# Autodesk Inventor assembly: Сборка част.-аналог.V3.0
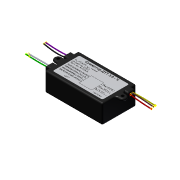
[picture p0: Inventor's stored thumbnail of the model, 180x180]
Saved by Autodesk Inventor 2012 (Build 160160000, 160)
## iProperties
Created: 2009-11-20
Part Number: Сборка част.-аналог.V3.0
Document SubType Name: Assembly
Designer: toma
Mass: 20.6369 g
Surface Area: 289.802 cm^2
Volume: 20.6369 cm^3
Density: 1 g/cm^3
Author: toma
## Documents named in this file (7)
- D:\VSS_WORK\VSS_ENERGO\Сумматор light\КД\Сумматор Light\Сумматор частотно-аналоговый\Сборка част.-аналог.V3.0.iam
- D:\VSS_WORK\VSS_ENERGO\Сумматор light\КД\Сумматор Light\корпус.ipt
- D:\VSS_WORK\VSS_ENERGO\Сумматор light\КД\Сумматор Light\клей.ipt
- D:\VSS_WORK\VSS_ENERGO\Сумматор light\КД\Сумматор Light\контакт.ipt
- D:\Inventor\Сумматор Light\Сборка2\AIP\Провода и кабели\Сборка2.Прокладка кабелей1.iam
- D:\VSS_WORK\VSS_ENERGO\Сумматор light\КД\Сумматор Light\Импортированные компоненты\Сумматор light частотно-аналоговый V3.0\Сумматор light частотно-аналоговый V3.0.iam
- D:\VSS_WORK\VSS_ENERGO\Сумматор light\КД\Сумматор Light\Сумматор частотно-аналоговый\крышка Ч_А.ipt
## Components (20 placed, 6 different names)
1. корпус:1 — Совмещение:4, Совмещение:5, Совмещение:6, Совмещение:8, Совмещение:9, Совмещение:10, Совмещение:11, Совмещение:12, Совмещение:13, Совмещение:14, Совмещение:17, Совмещение:18, Совмещение:19, Совмещение:20, Совмещение:21, Совмещение:22, Совмещение:23, Совмещение:24, Совмещение:25, Совмещение:26, Совмещение:27, Совмещение:28, Совмещение:38, Совмещение:41, Совмещение:42, Совмещение:43, Совмещение:44, Совмещение:45, Совмещение:47, Совмещение:48, Совмещение:49
2. клей:1 — Совмещение:4, Совмещение:39, Совмещение:40, Совмещение:41, Совмещение:42
3. контакт:1 — Совмещение:5, Совмещение:6, Совмещение:11
4. контакт:2 — Совмещение:8, Совмещение:9, Совмещение:10
5. контакт:3 — Совмещение:12, Совмещение:13, Совмещение:14
6. контакт:4 — Совмещение:18, Совмещение:19, Совмещение:20
7. контакт:5 — Совмещение:17, Совмещение:21, Совмещение:22
8. контакт:6 — Совмещение:23, Совмещение:24, Совмещение:25
9. контакт:7 — Совмещение:26, Совмещение:27, Совмещение:28
10. Прокладка кабелей1 [sub-assembly]
11. Сумматор light частотно-аналоговый V3.0:1 [sub-assembly] — Совмещение:38, Совмещение:39, Совмещение:40
12. контакт:8
13. контакт:9
14. контакт:10
15. контакт:11
16. контакт:12
17. контакт:13
18. контакт:14
19. контакт:15 — Совмещение:43, Совмещение:44, Совмещение:45
20. крышка Ч_А:1 — Совмещение:47, Совмещение:48, Совмещение:49
## Relationships (33: Mate 33)
- Совмещение:4 [Mate]: корпус:1 ↔ клей:1
- Совмещение:5 [Mate] (25 mm): корпус:1 ↔ контакт:1
- Совмещение:6 [Mate] (0.5 mm): корпус:1 ↔ контакт:1
- Совмещение:8 [Mate] (25 mm): корпус:1 ↔ контакт:2
- Совмещение:9 [Mate] (1.5 mm): корпус:1 ↔ контакт:2
- Совмещение:10 [Mate] (1.8 mm): корпус:1 ↔ контакт:2
- Совмещение:11 [Mate] (-0.5 mm): корпус:1 ↔ контакт:1
- Совмещение:12 [Mate] (25 mm): корпус:1 ↔ контакт:3
- Совмещение:13 [Mate] (1.5 mm): корпус:1 ↔ контакт:3
- Совмещение:14 [Mate] (4.3 mm): корпус:1 ↔ контакт:3
- Совмещение:17 [Mate] (3.2 mm): корпус:1 ↔ контакт:5
- Совмещение:18 [Mate] (1.5 mm): корпус:1 ↔ контакт:4
- Совмещение:19 [Mate] (1.2 mm): корпус:1 ↔ контакт:4
- Совмещение:20 [Mate] (25 mm): корпус:1 ↔ контакт:4
- Совмещение:21 [Mate] (1.5 mm): корпус:1 ↔ контакт:5
- Совмещение:22 [Mate] (25 mm): корпус:1 ↔ контакт:5
- Совмещение:23 [Mate] (24 mm): корпус:1 ↔ контакт:6
- Совмещение:24 [Mate] (1.5 mm): корпус:1 ↔ контакт:6
- Совмещение:25 [Mate] (1.5 mm): корпус:1 ↔ контакт:6
- Совмещение:26 [Mate] (25 mm): корпус:1 ↔ контакт:7
- Совмещение:27 [Mate] (1.5 mm): корпус:1 ↔ контакт:7
- Совмещение:28 [Mate] (3.5 mm): корпус:1 ↔ контакт:7
- Совмещение:38 [Mate] (2.5 mm): корпус:1 ↔ Сумматор light частотно-аналоговый V3.0:1
- Совмещение:39 [Mate]: клей:1 ↔ Сумматор light частотно-аналоговый V3.0:1
- Совмещение:40 [Mate]: клей:1 ↔ Сумматор light частотно-аналоговый V3.0:1
- Совмещение:41 [Mate]: корпус:1 ↔ клей:1
- Совмещение:42 [Mate]: корпус:1 ↔ клей:1
- Совмещение:43 [Mate] (25 mm): корпус:1 ↔ контакт:15
- Совмещение:44 [Mate] (0.8 mm): корпус:1 ↔ контакт:15
- Совмещение:45 [Mate] (2 mm): корпус:1 ↔ контакт:15
- Совмещение:47 [Mate]: корпус:1 ↔ крышка Ч_А:1
- Совмещение:48 [Mate]: корпус:1 ↔ крышка Ч_А:1
- Совмещение:49 [Mate]: корпус:1 ↔ крышка Ч_А:1
